# Autodesk Inventor assembly: Header
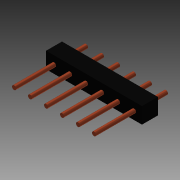
[picture p0: Inventor's stored thumbnail of the model, 180x180]
Saved by Autodesk Inventor 2013 (Build 170138000, 138)
## iProperties
Created: 2013-07-31
Part Number: Header
Document SubType Name: Assembly
Designer: Kyle
Author: Kyle
## Documents named in this file (3)
- C:\Users\Kyle\Documents\Inventor\2013\ROV\Motor Driver\Header.iam
- C:\Users\Kyle\Documents\Inventor\2013\ROV\Motor Driver\Main Header.ipt
- C:\Users\Kyle\Documents\Inventor\2013\ROV\Motor Driver\Header Pin.ipt
## Components (7 placed, 2 different names)
1. Main Header:1 — Mate:1, Mate:2, Mate:3, Mate:4, Mate:5, Mate:6, Flush:1, Flush:2, Flush:3, Flush:4, Flush:5, Flush:6
2. Header Pin:1 — Mate:1, Flush:6
3. Header Pin:2 — Mate:2, Flush:5
4. Header Pin:3 — Mate:3, Flush:4
5. Header Pin:4 — Mate:4, Flush:3
6. Header Pin:5 — Mate:6, Flush:1
7. Header Pin:6 — Mate:5, Flush:2
## Relationships (12: Mate 6, Flush 6)
- Mate:1: Main Header:1 ↔ Header Pin:1
- Mate:2: Main Header:1 ↔ Header Pin:2
- Mate:3: Main Header:1 ↔ Header Pin:3
- Mate:4: Main Header:1 ↔ Header Pin:4
- Mate:5: Main Header:1 ↔ Header Pin:6
- Mate:6: Main Header:1 ↔ Header Pin:5
- Flush:1 (-6.35 mm): Main Header:1 ↔ Header Pin:5
- Flush:2 (-6.35 mm): Main Header:1 ↔ Header Pin:6
- Flush:3 (-6.35 mm): Main Header:1 ↔ Header Pin:4
- Flush:4 (-6.35 mm): Main Header:1 ↔ Header Pin:3
- Flush:5 (-6.35 mm): Main Header:1 ↔ Header Pin:2
- Flush:6 (-6.35 mm): Main Header:1 ↔ Header Pin:1
